# Autodesk Inventor assembly: asm_mate
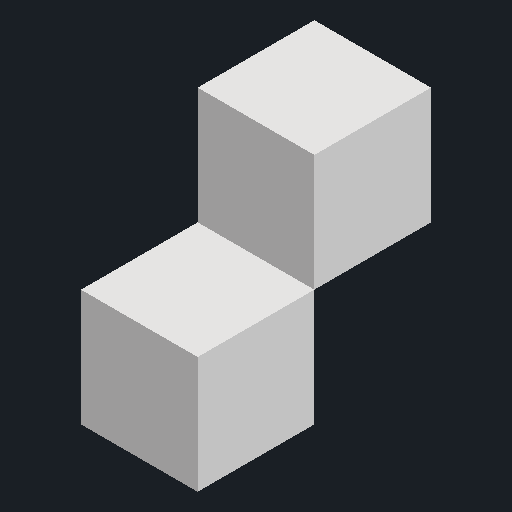
[picture p0: Inventor's stored thumbnail of the model, 512x512]
Saved by Autodesk Inventor 2027 (Build 310192060, 192F)
## iProperties
Created: 2026-07-12
Part Number: asm_mate
Document SubType Name: Assembly
Designer: vmiguel
Author: vmiguel
## Documents named in this file (2)
- C:\Users\vmiguel\git\oblikovati-workspace\_iptformat\corpus\asm_mate.iam
- C:\Users\vmiguel\git\oblikovati-workspace\_iptformat\corpus\asm_cube.ipt
## Components (2 placed, 1 different names)
1. asm_cube:1 — Mate:1
2. asm_cube:2 — Mate:1
## Relationships (1: Mate 1)
- Mate:1: asm_cube:1 ↔ asm_cube:2
